# Autodesk Inventor assembly: rjPack
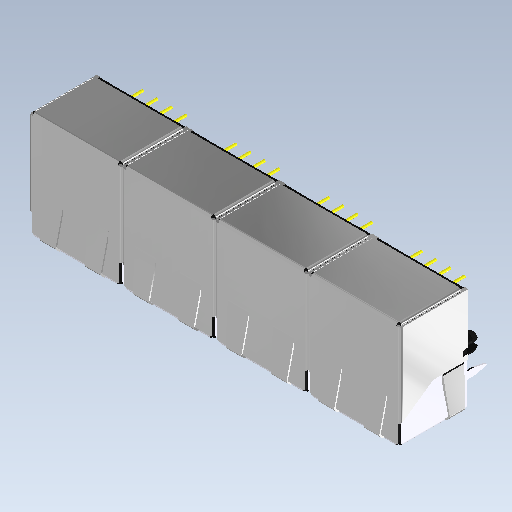
[picture p0: Inventor's stored thumbnail of the model, 512x512]
Saved by Autodesk Inventor 2021 (Build 250183000, 183)
## iProperties
Created: 2023-08-06
Part Number: rjPack
Document SubType Name: Assembly
Designer: michal
Author: michal
## Documents named in this file (2)
- C:\Users\micha\OneDrive\Dokumenty\GitHub\escape_room_hw_v2\Enclosure\Commercial\rjPack.iam
- C:\Users\micha\OneDrive\Dokumenty\GitHub\escape_room_hw_v2\Enclosure\Commercial\139341875-9-2-338556-1\2-338556-1.ipt
## Components (4 placed, 1 different names)
1. 2-338556-1:1
2. 2-338556-1:2
3. 2-338556-1:3
4. 2-338556-1:4
## Relationships (9: Flush 6, Mate 3)
- [Flush]: 2-338556-1:1 ↔ 2-338556-1:2
- [Flush]: 2-338556-1:2 ↔ 2-338556-1:3
- [Flush]: 2-338556-1:3 ↔ 2-338556-1:4
- [Mate]: 2-338556-1:1 ↔ 2-338556-1:2
- [Mate]: 2-338556-1:2 ↔ 2-338556-1:3
- [Mate]: 2-338556-1:3 ↔ 2-338556-1:4
- [Flush]: 2-338556-1:1 ↔ 2-338556-1:2
- [Flush]: 2-338556-1:2 ↔ 2-338556-1:3
- [Flush]: 2-338556-1:3 ↔ 2-338556-1:4
